# Autodesk Inventor assembly: prototype for arm
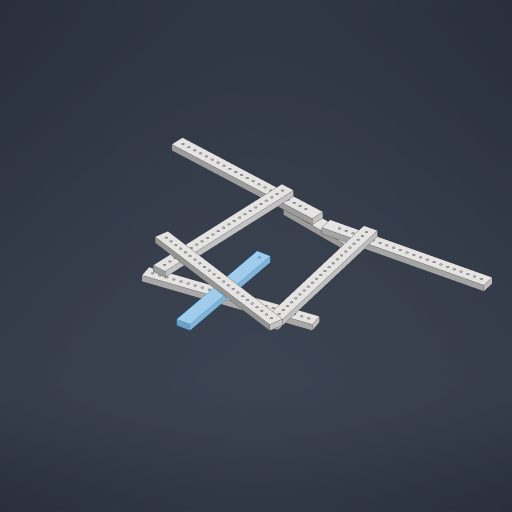
[picture p0: Inventor's stored thumbnail of the model, 512x512]
Saved by Autodesk Inventor 2023 (Build 270158000, 158)
## iProperties
Created: 2023-01-24
Part Number: prototype for arm
Document SubType Name: Assembly
Designer: Blank Slate
Author: Blank Slate
## Documents named in this file (5)
- C:\Users\bryce\Downloads\FRC_2023_saberdynamics-main\FRC_2023_saberdynamics-main\prototype for arm.iam
- C:\Users\bryce\Downloads\FRC_2023_saberdynamics-main\FRC_2023_saberdynamics-main\pincer2.0.ipt
- C:\Users\bryce\Downloads\FRC_2023_saberdynamics-main\FRC_2023_saberdynamics-main\flat.ipt
- C:\Users\bryce\Downloads\FRC_2023_saberdynamics-main\FRC_2023_saberdynamics-main\linkage.ipt
- C:\Users\bryce\Downloads\FRC_2023_saberdynamics-main\FRC_2023_saberdynamics-main\track.ipt
## Components (8 placed, 4 different names)
1. pincer2.0:1 — Insert:2, Insert:9, Flush:1
2. pincer2.0:2 — Insert:1, Insert:10, Flush:2
3. flat:1 — Insert:1, Insert:2
4. linkage:3 — Insert:10, Flush:2, Insert:11
5. joint — Insert:7, Insert:8
6. linkage:4 — Insert:9, Flush:1, Insert:12
7. linkage:5 — Insert:7, Insert:11
8. linkage:6 — Insert:8, Insert:12
## Relationships (10: Insert 8, Flush 2)
- Insert:1: pincer2.0:2 ↔ flat:1
- Insert:2: pincer2.0:1 ↔ flat:1
- Insert:7: joint ↔ linkage:5
- Insert:8: joint ↔ linkage:6
- Insert:9: pincer2.0:1 ↔ linkage:4
- Insert:10: pincer2.0:2 ↔ linkage:3
- Flush:1: pincer2.0:1 ↔ linkage:4
- Flush:2: pincer2.0:2 ↔ linkage:3
- Insert:11: linkage:3 ↔ linkage:5
- Insert:12: linkage:4 ↔ linkage:6
